# Autodesk Inventor assembly: wahaczserwo
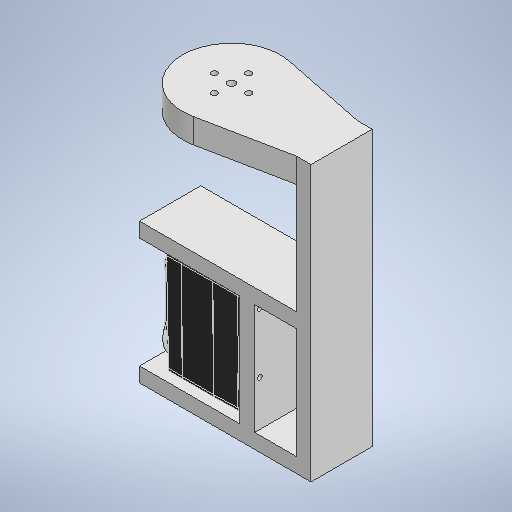
[picture p0: Inventor's stored thumbnail of the model, 512x512]
Saved by Autodesk Inventor 2025.3 (Build 293356000, 356)
## iProperties
Created: 2026-03-20
Part Number: wahaczserwo
Document SubType Name: Assembly
Designer: ksawe
Author: ksawe
## Documents named in this file (3)
- C:\Users\ksawe\OneDrive\Pulpit\Exomy v1\wahaczserwo.iam
- C:\Users\ksawe\OneDrive\Pulpit\Exomy v1\wahacz.ipt
- C:\Users\ksawe\OneDrive\Pulpit\Exomy v1\ST3215\ST3215\ST3215.iam
## Components (2 placed, 2 different names)
1. wahacz:1 — Mate:1
2. ST3215:1 [sub-assembly] — Mate:1
## Relationships (1: Mate 1)
- Mate:1: wahacz:1 ↔ ST3215:1
